# Autodesk Inventor assembly: DisplayDummyAuschnitt
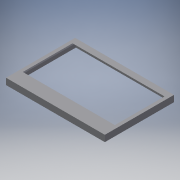
[picture p0: Inventor's stored thumbnail of the model, 180x180]
Saved by Autodesk Inventor 2017 SP1 (Build 210196100, 196)
## iProperties
Part Number: DisplayDummyAuschnitt
Material: Generisch
Document SubType Name: Assembly
Designer: aXe
Author: aXe
## Documents named in this file (4)
- C:\Users\aXe\Dropbox\Elektronik\aXe_Dashboard240XL\Gehäuse\DisplayDummyAuschnitt.iam
- C:\Users\aXe\Dropbox\Elektronik\aXe_Dashboard240XL\Gehäuse\DisplayDummy.ipt
- C:\Users\aXe\Dropbox\Elektronik\aXe_Dashboard240XL\Gehäuse\DummyAuschnitt.ipt
- C:\Users\aXe\Dropbox\Elektronik\aXe_Dashboard240XL\Gehäuse\Auschnitt2.ipt
## Components (3 placed, 3 different names)
1. DisplayDummy:1 — Fluchtend:1, Fluchtend:2, Fluchtend:3, Fluchtend:4, Fluchtend:5
2. DummyAuschnitt:1 — Fluchtend:1, Fluchtend:2, Fluchtend:3
3. Auschnitt2:1 — Fluchtend:4, Fluchtend:5
## Relationships (5: Flush 5)
- Fluchtend:1 [Flush]: DisplayDummy:1 ↔ DummyAuschnitt:1
- Fluchtend:2 [Flush]: DisplayDummy:1 ↔ DummyAuschnitt:1
- Fluchtend:3 [Flush]: DisplayDummy:1 ↔ DummyAuschnitt:1
- Fluchtend:4 [Flush]: DisplayDummy:1 ↔ Auschnitt2:1
- Fluchtend:5 [Flush]: DisplayDummy:1 ↔ Auschnitt2:1
